# Autodesk Inventor assembly: SEPARACION LATA-BOTELLA Y PAPEL
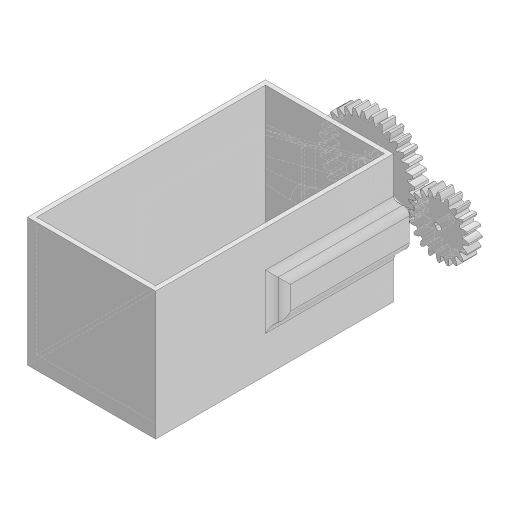
[picture p0: Inventor's stored thumbnail of the model, 512x512]
Saved by Autodesk Inventor 2024 (Build 280153000, 153)
## iProperties
Created: 2024-06-16
Part Number: SEPARACION LATA-BOTELLA Y PAPEL
Document SubType Name: Assembly
Designer: Jhuliams
Author: Jhuliams
## Documents named in this file (4)
- C:\Users\Jhuliams\Documents\GitHub\RECICLADOR_MODELO_3D\MECANISMO DE COMPACTADO\SEPARACION LATA-BOTELLA Y PAPEL.iam
- C:\Users\Jhuliams\Documents\GitHub\RECICLADOR_MODELO_3D\MECANISMO DE COMPACTADO\CAJA PARA DETECCION DE OBJETO.ipt
- C:\Users\Jhuliams\Documents\GitHub\RECICLADOR_MODELO_3D\MECANISMO DE COMPACTADO\ENGRANAJE CONDUCTOR DE CAJA.ipt
- C:\Users\Jhuliams\Documents\GitHub\RECICLADOR_MODELO_3D\MECANISMO DE COMPACTADO\ENGRANE MOTRIZ DE CAJA.ipt
## Components (3 placed, 3 different names)
1. CAJA PARA DETECCION DE OBJETO:1 — Mate:3, Flush:2, Flush:3
2. ENGRANAJE CONDUCTOR DE CAJA:1 — Flush:1, Mate:2, Mate:3, Flush:2, Rotation:1, Flush:3
3. ENGRANE MOTRIZ DE CAJA:1 — Mate:1, Flush:1, Mate:2, Rotation:1
## Relationships (7: Mate 3, Flush 3, RelateRotation 1)
- Mate:1: ENGRANE MOTRIZ DE CAJA:1
- Flush:1: ENGRANAJE CONDUCTOR DE CAJA:1 ↔ ENGRANE MOTRIZ DE CAJA:1
- Mate:2 (79.5 mm): ENGRANAJE CONDUCTOR DE CAJA:1 ↔ ENGRANE MOTRIZ DE CAJA:1
- Mate:3: CAJA PARA DETECCION DE OBJETO:1 ↔ ENGRANAJE CONDUCTOR DE CAJA:1
- Flush:2: CAJA PARA DETECCION DE OBJETO:1 ↔ ENGRANAJE CONDUCTOR DE CAJA:1
- Rotation:1 [RelateRotation] (1.65 ul): ENGRANAJE CONDUCTOR DE CAJA:1 ↔ ENGRANE MOTRIZ DE CAJA:1
- Flush:3: CAJA PARA DETECCION DE OBJETO:1 ↔ ENGRANAJE CONDUCTOR DE CAJA:1
